# Autodesk Inventor assembly: MiniPad
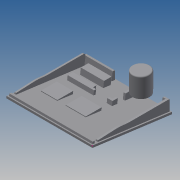
[picture p0: Inventor's stored thumbnail of the model, 180x180]
Saved by Autodesk Inventor 2019 (Build 230136000, 136)
## iProperties
Created: 2022-10-27
Part Number: MiniPad
Material: Generisch
Document SubType Name: Assembly
Designer: Dominik Schmidt
Author: Dominik Schmidt
## Documents named in this file (5)
- C:\Users\Dominik Schmidt\Desktop\DIY Mini Keypad\MiniPad.iam
- C:\Users\Dominik Schmidt\Desktop\DIY Mini Keypad\Top.ipt
- C:\Users\Dominik Schmidt\Desktop\DIY Mini Keypad\Bottom.ipt
- C:\Users\Dominik Schmidt\Desktop\DIY Mini Keypad\Tastatur.ipt
- C:\Users\Dominik Schmidt\Desktop\DIY Mini Keypad\Knopp.ipt
## Components (4 placed, 4 different names)
1. Top:1 — Fluchtend:1, Fluchtend:2, Fluchtend:3
2. Bottom:1 — Fluchtend:1
3. Tastatur:1 — Fluchtend:2
4. Knopp:1 — Fluchtend:3
## Relationships (3: Flush 3)
- Fluchtend:1 [Flush]: Top:1 ↔ Bottom:1
- Fluchtend:2 [Flush]: Top:1 ↔ Tastatur:1
- Fluchtend:3 [Flush]: Top:1 ↔ Knopp:1
